# Autodesk Inventor assembly: Beam_v3
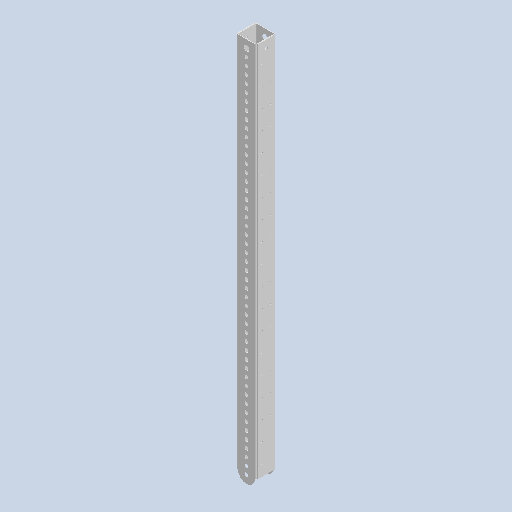
[picture p0: Inventor's stored thumbnail of the model, 512x512]
Saved by Autodesk Inventor 2022 (Build 260153000, 153)
## iProperties
Created: 2022-04-25
Part Number: Beam_v3
Document SubType Name: Assembly
Designer: Patrick
Author: Patrick
## Documents named in this file (3)
- C:\Users\patri\OneDrive - Syddansk Universitet\2. Semester Master\Mekaniske Elementer\Mini Project\2020-10-23\Workspaces\Workspace\Beam\Beam_v3.iam
- C:\Users\patri\OneDrive - Syddansk Universitet\2. Semester Master\Mekaniske Elementer\Mini Project\2020-10-23\Workspaces\Workspace\Beam\HalvBeam_V3.ipt
- C:\Users\patri\OneDrive - Syddansk Universitet\2. Semester Master\Mekaniske Elementer\Mini Project\2020-10-23\Workspaces\Workspace\Beam\Assembly_plate_beamV3.ipt
## Components (4 placed, 2 different names)
1. HalvBeam_V3:1 — Rigid:1, Rigid:3
2. HalvBeam_V3:2 — Rigid:1, Rigid:2
3. Assembly_plate_beamV3:1 — Rigid:3
4. Assembly_plate_beamV3:2 — Rigid:2
## Relationships (3: WeldJoint 3)
- Rigid:1 [WeldJoint]: HalvBeam_V3:1 ↔ HalvBeam_V3:2
- Rigid:2 [WeldJoint]: HalvBeam_V3:2 ↔ Assembly_plate_beamV3:2
- Rigid:3 [WeldJoint]: HalvBeam_V3:1 ↔ Assembly_plate_beamV3:1
